# Autodesk Inventor assembly: BevelPlate_Prep
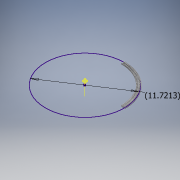
[picture p0: Inventor's stored thumbnail of the model, 180x180]
Saved by Autodesk Inventor 2017 (Build 210142000, 142)
## iProperties
Created: 2017-01-26
Part Number: BevelPlate_Prep
Document SubType Name: Assembly
Designer: David Kopala
Author: David Kopala
## Documents named in this file (4)
- Z:\Documents\Drone\Drone\3D Models\Project\Chassis_04\PrinterStaging\BevelPlate_Prep.iam
- Z:\Documents\Drone\Drone\3D Models\Project\Chassis_04\BevelBasePlate.ipt
- Z:\Documents\Drone\Drone\3D Models\Project\Chassis_04\BevelGear_Ref\Design Accelerator\Bevel Gear13.ipt
- Z:\Documents\Drone\Drone\3D Models\Project\Chassis_04\BevelOuter_Ref\Design Accelerator\Bevel Gear11.ipt
## Components (3 placed, 2 different names)
1. BevelBasePlate:1 — Insert:1
2. Bevel Gear1:1 — Insert:1, Insert:2
3. Bevel Gear1:2 — Insert:2
## Relationships (2: Insert 2)
- Insert:1: BevelBasePlate:1 ↔ Bevel Gear1:1
- Insert:2: Bevel Gear1:1 ↔ Bevel Gear1:2
